# Autodesk Inventor assembly: Assembly finished robot ver22
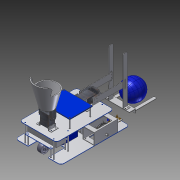
[picture p0: Inventor's stored thumbnail of the model, 180x180]
Saved by Autodesk Inventor 2015 (Build 190159000, 159)
## iProperties
Created: 2015-05-24
Part Number: Assembly finished robot ver22
Document SubType Name: Assembly
Designer: kenta
Mass: 1326.89 g
Surface Area: 4695.11 cm^2
Volume: 1106.31 cm^3
Density: 1.19938 g/cm^3
Author: kenta
## Documents named in this file (26)
- C:\Users\kenta\Documents\Inventor\知能ロボコン\Assembly finished robot ver2.1.iam
- C:\Users\kenta\Documents\Inventor\知能ロボコン\Board 1.ipt
- C:\Users\kenta\Documents\Inventor\知能ロボコン\Caster board.ipt
- C:\Users\kenta\Documents\Inventor\知能ロボコン\Caster pole 1.ipt
- C:\Users\kenta\Documents\Inventor\知能ロボコン\Caster.ipt
- C:\Users\kenta\Documents\Inventor\知能ロボコン\Board 2.ipt
- C:\Users\kenta\Documents\Inventor\知能ロボコン\PSD catch.ipt
- C:\Users\kenta\Documents\Inventor\知能ロボコン\Caster pole 2.ipt
- C:\Users\kenta\Documents\Inventor\知能ロボコン\Servo catch back.ipt
- C:\Users\kenta\Documents\Inventor\知能ロボコン\Servo catch front.ipt
- C:\Users\kenta\Documents\Inventor\知能ロボコン\Servo neck.ipt
- C:\Users\kenta\Documents\Inventor\知能ロボコン\Servo KRS-2542HV ICS.ipt
- C:\Users\kenta\Documents\Inventor\知能ロボコン\PSD sensor.ipt
- C:\Users\kenta\Documents\Inventor\知能ロボコン\Line trace.ipt
- C:\Users\kenta\Documents\Inventor\知能ロボコン\Battery.ipt
- C:\Users\kenta\Documents\Inventor\知能ロボコン\Assembly bottom ver2.iam
- C:\Users\kenta\Documents\Inventor\知能ロボコン\Fork ver2\Assembly fork ver2.iam
- C:\Users\kenta\Documents\Inventor\知能ロボコン\Nut.ipt
- C:\Users\kenta\Documents\Inventor\知能ロボコン\Line trace catch.ipt
- C:\Users\kenta\Documents\Inventor\知能ロボコン\Screw_20mm.ipt
- C:\Users\kenta\Documents\Inventor\知能ロボコン\Screw_10mm.ipt
- C:\Users\kenta\Documents\Inventor\知能ロボコン\Ball bule.ipt
- C:\Users\kenta\Documents\Inventor\知能ロボコン\Main board ver2.ipt
- C:\Users\kenta\Documents\Inventor\知能ロボコン\Motor board ver2.ipt
- C:\Users\kenta\Documents\Inventor\知能ロボコン\Ball saucer.ipt
- C:\Users\kenta\Documents\Inventor\知能ロボコン\LineTraceCoverFlont.ipt
## Components (63 placed, 25 different names)
1. Board 1:1 — メイト:1, 挿入:17, 挿入:18, 挿入:19, 挿入:20, 挿入:23, 挿入:24, 挿入:30, 挿入:31, 挿入:32, 挿入:33, 挿入:64, 挿入:65, 挿入:66, 挿入:67, 挿入:83, 挿入:84, 挿入:85, 挿入:86, 挿入:87, 挿入:89, 挿入:91, 挿入:93, 挿入:107, 挿入:108, 挿入:109, 挿入:110, 挿入:129, 挿入:130
2. Caster board:1 — 挿入:21, 挿入:22, 挿入:25, 挿入:26, 挿入:27, メイト:7
3. Caster pole 1:1 — 挿入:17, 挿入:21
4. Caster pole 1:2 — 挿入:18, 挿入:22
5. Caster pole 1:3 — 挿入:19
6. Caster pole 1:4 — 挿入:20
7. Caster:1 — 挿入:25, 挿入:26, 挿入:27
8. Board 2:1 — 挿入:28, 挿入:29, 挿入:68, 挿入:70, 挿入:72, 挿入:74, 挿入:79, 挿入:123, 挿入:124, 挿入:125, 挿入:126
9. PSD catch:1 — 挿入:23, 挿入:24, 挿入:28, 挿入:29, メイト:3
10. Caster pole 2:1 — 挿入:30
11. Caster pole 2:2 — 挿入:31
12. Caster pole 2:3 — 挿入:32
13. Caster pole 2:4 — 挿入:33
14. Servo catch back:1 — 挿入:68, 挿入:69
15. Servo catch back:2 — 挿入:70, 挿入:71, 挿入:72, 挿入:73
16. Servo catch front:2 — 挿入:74, 挿入:75, 挿入:76
17. Servo catch front:1 — 挿入:77, 挿入:78, 挿入:79
18. Servo neck:1 — 挿入:42, 挿入:131
19. Servo neck:2 — 挿入:80, 挿入:81, 挿入:82
20. Servo KRS-2542HV ICS:1 — 挿入:75, 挿入:76, 挿入:77, 挿入:78, 挿入:80
21. Servo KRS-2542HV ICS:2 — 挿入:42, 挿入:69, 挿入:71, 挿入:73
22. PSD sensor:1 — メイト:3
23. Line trace:1 — 挿入:120, 挿入:121, 挿入:122, 挿入:132, 挿入:133
24. Battery:1 — メイト:7
25. Assembly bottom ver2:1 [sub-assembly] — 挿入:64, 挿入:65, 挿入:83, 挿入:84
26. Assembly bottom ver2:2 [sub-assembly] — 挿入:66, 挿入:67, 挿入:85, 挿入:86
27. Assembly fork ver2:1 [sub-assembly] — 挿入:81, 挿入:82
28. Nut:1 — 挿入:87, 挿入:88
29. Nut:2 — 挿入:88, 挿入:95
30. Nut:3 — 挿入:89, 挿入:90
31. Nut:4 — 挿入:90, 挿入:96
32. Nut:5 — 挿入:94, 挿入:98
33. Nut:6 — 挿入:93, 挿入:94
34. Nut:7 — 挿入:92, 挿入:97
35. Nut:8 — 挿入:91, 挿入:92
36. Line trace catch:1 — 挿入:95, 挿入:96, 挿入:103, 挿入:104, 挿入:111, 挿入:112
37. Line trace catch:2 — 挿入:97, 挿入:98, 挿入:105, 挿入:106, 挿入:113, 挿入:114
38. Screw_20mm:2 — 挿入:120
39. Screw_20mm:3 — 挿入:115, 挿入:121
40. Screw_20mm:4 — 挿入:122
41. Nut:9 — 挿入:103, 挿入:115
42. Nut:10 — 挿入:104
43. Nut:11 — 挿入:105
44. Nut:12 — 挿入:106
45. Screw_10mm:1 — 挿入:107
46. Screw_10mm:2 — 挿入:108
47. Screw_10mm:3 — 挿入:109
48. Screw_10mm:4 — 挿入:110
49. Nut:13 — 挿入:111
50. Nut:14 — 挿入:112
51. Nut:15 — 挿入:113
52. Nut:16 — 挿入:114
53. Nut:17
54. Ball bule:1
55. Caster pole 1:5 — 挿入:123, 挿入:127
56. Caster pole 1:6 — 挿入:124, 挿入:128
57. Caster pole 1:7 — 挿入:126
58. Caster pole 1:8 — 挿入:125
59. Main board ver2:1 — 挿入:127, 挿入:128
60. Motor board ver2:1 — 挿入:129, 挿入:130
61. Ball saucer:1 — 挿入:131
62. Screw_20mm:5 — 挿入:134
63. LineTraceCoverFlont:1 — 挿入:132, 挿入:133, 挿入:134
## Relationships (84: Insert 81, Mate 3)
- メイト:1 [Mate]: Board 1:1
- 挿入:17 [Insert]: Board 1:1 ↔ Caster pole 1:1
- 挿入:18 [Insert]: Board 1:1 ↔ Caster pole 1:2
- 挿入:19 [Insert]: Board 1:1 ↔ Caster pole 1:3
- 挿入:20 [Insert]: Board 1:1 ↔ Caster pole 1:4
- 挿入:21 [Insert]: Caster board:1 ↔ Caster pole 1:1
- 挿入:22 [Insert]: Caster board:1 ↔ Caster pole 1:2
- 挿入:23 [Insert]: Board 1:1 ↔ PSD catch:1
- 挿入:24 [Insert]: Board 1:1 ↔ PSD catch:1
- 挿入:25 [Insert]: Caster board:1 ↔ Caster:1
- 挿入:26 [Insert]: Caster board:1 ↔ Caster:1
- 挿入:27 [Insert]: Caster board:1 ↔ Caster:1
- 挿入:28 [Insert]: Board 2:1 ↔ PSD catch:1
- 挿入:29 [Insert]: Board 2:1 ↔ PSD catch:1
- 挿入:30 [Insert]: Board 1:1 ↔ Caster pole 2:1
- 挿入:31 [Insert]: Board 1:1 ↔ Caster pole 2:2
- 挿入:32 [Insert]: Board 1:1 ↔ Caster pole 2:3
- 挿入:33 [Insert]: Board 1:1 ↔ Caster pole 2:4
- 挿入:42 [Insert]: Servo neck:1 ↔ Servo KRS-2542HV ICS:2
- メイト:3 [Mate]: PSD catch:1 ↔ PSD sensor:1
- メイト:7 [Mate]: Caster board:1 ↔ Battery:1
- 挿入:64 [Insert]: Board 1:1 ↔ Assembly bottom ver2:1
- 挿入:65 [Insert]: Board 1:1 ↔ Assembly bottom ver2:1
- 挿入:66 [Insert]: Board 1:1 ↔ Assembly bottom ver2:2
- 挿入:67 [Insert]: Board 1:1 ↔ Assembly bottom ver2:2
- 挿入:68 [Insert]: Board 2:1 ↔ Servo catch back:1
- 挿入:69 [Insert]: Servo catch back:1 ↔ Servo KRS-2542HV ICS:2
- 挿入:70 [Insert]: Board 2:1 ↔ Servo catch back:2
- 挿入:71 [Insert]: Servo catch back:2 ↔ Servo KRS-2542HV ICS:2
- 挿入:72 [Insert]: Board 2:1 ↔ Servo catch back:2
- 挿入:73 [Insert]: Servo catch back:2 ↔ Servo KRS-2542HV ICS:2
- 挿入:74 [Insert]: Board 2:1 ↔ Servo catch front:2
- 挿入:75 [Insert]: Servo catch front:2 ↔ Servo KRS-2542HV ICS:1
- 挿入:76 [Insert]: Servo catch front:2 ↔ Servo KRS-2542HV ICS:1
- 挿入:77 [Insert]: Servo catch front:1 ↔ Servo KRS-2542HV ICS:1
- 挿入:78 [Insert]: Servo catch front:1 ↔ Servo KRS-2542HV ICS:1
- 挿入:79 [Insert]: Board 2:1 ↔ Servo catch front:1
- 挿入:80 [Insert]: Servo neck:2 ↔ Servo KRS-2542HV ICS:1
- 挿入:81 [Insert]: Servo neck:2 ↔ Assembly fork ver2:1
- 挿入:82 [Insert]: Servo neck:2 ↔ Assembly fork ver2:1
- 挿入:83 [Insert]: Board 1:1 ↔ Assembly bottom ver2:1
- 挿入:84 [Insert]: Board 1:1 ↔ Assembly bottom ver2:1
- 挿入:85 [Insert]: Board 1:1 ↔ Assembly bottom ver2:2
- 挿入:86 [Insert]: Board 1:1 ↔ Assembly bottom ver2:2
- 挿入:87 [Insert]: Board 1:1 ↔ Nut:1
- 挿入:88 [Insert]: Nut:1 ↔ Nut:2
- 挿入:89 [Insert]: Board 1:1 ↔ Nut:3
- 挿入:90 [Insert]: Nut:3 ↔ Nut:4
- 挿入:91 [Insert]: Board 1:1 ↔ Nut:8
- 挿入:92 [Insert]: Nut:7 ↔ Nut:8
- 挿入:93 [Insert]: Board 1:1 ↔ Nut:6
- 挿入:94 [Insert]: Nut:5 ↔ Nut:6
- 挿入:95 [Insert]: Nut:2 ↔ Line trace catch:1
- 挿入:96 [Insert]: Nut:4 ↔ Line trace catch:1
- 挿入:97 [Insert]: Nut:7 ↔ Line trace catch:2
- 挿入:98 [Insert]: Nut:5 ↔ Line trace catch:2
- 挿入:103 [Insert]: Line trace catch:1 ↔ Nut:9
- 挿入:104 [Insert]: Line trace catch:1 ↔ Nut:10
- 挿入:105 [Insert]: Line trace catch:2 ↔ Nut:11
- 挿入:106 [Insert]: Line trace catch:2 ↔ Nut:12
- 挿入:107 [Insert]: Board 1:1 ↔ Screw_10mm:1
- 挿入:108 [Insert]: Board 1:1 ↔ Screw_10mm:2
- 挿入:109 [Insert]: Board 1:1 ↔ Screw_10mm:3
- 挿入:110 [Insert]: Board 1:1 ↔ Screw_10mm:4
- 挿入:111 [Insert]: Line trace catch:1 ↔ Nut:13
- 挿入:112 [Insert]: Line trace catch:1 ↔ Nut:14
- 挿入:113 [Insert]: Line trace catch:2 ↔ Nut:15
- 挿入:114 [Insert]: Line trace catch:2 ↔ Nut:16
- 挿入:115 [Insert] (-5 mm): Screw_20mm:3 ↔ Nut:9
- 挿入:120 [Insert] (1 mm): Line trace:1 ↔ Screw_20mm:2
- 挿入:121 [Insert] (1 mm): Line trace:1 ↔ Screw_20mm:3
- 挿入:122 [Insert] (1 mm): Line trace:1 ↔ Screw_20mm:4
- 挿入:123 [Insert]: Board 2:1 ↔ Caster pole 1:5
- 挿入:124 [Insert]: Board 2:1 ↔ Caster pole 1:6
- 挿入:125 [Insert]: Board 2:1 ↔ Caster pole 1:8
- 挿入:126 [Insert]: Board 2:1 ↔ Caster pole 1:7
- 挿入:127 [Insert]: Caster pole 1:5 ↔ Main board ver2:1
- 挿入:128 [Insert]: Caster pole 1:6 ↔ Main board ver2:1
- 挿入:129 [Insert]: Board 1:1 ↔ Motor board ver2:1
- 挿入:130 [Insert]: Board 1:1 ↔ Motor board ver2:1
- 挿入:131 [Insert]: Servo neck:1 ↔ Ball saucer:1
- 挿入:132 [Insert]: Line trace:1 ↔ LineTraceCoverFlont:1
- 挿入:133 [Insert]: Line trace:1 ↔ LineTraceCoverFlont:1
- 挿入:134 [Insert]: Screw_20mm:5 ↔ LineTraceCoverFlont:1
